# Autodesk Inventor assembly: ModuleBase
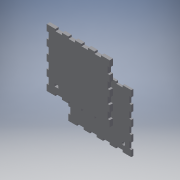
[picture p0: Inventor's stored thumbnail of the model, 180x180]
Saved by Autodesk Inventor 2019.4 (Build 234330000, 330)
## iProperties
Created: 2020-06-30
Part Number: ModuleBase
Document SubType Name: Assembly
Designer: wimva
Author: wimva
## Documents named in this file (4)
- C:\Users\wimva\source\repos\BombSquad\Mechanical\Modules\ModuleBase.iam
- C:\Users\wimva\source\repos\BombSquad\Mechanical\Modules\FrontPlateBase.ipt
- C:\Users\wimva\source\repos\BombSquad\Mechanical\Modules\BackPlateBase.ipt
- C:\Users\wimva\source\repos\BombSquad\Mechanical\Modules\Dimensions.xlsx
## Components (2 placed, 2 different names)
1. FrontPlateBase:1
2. BackPlateBase:1
## Named parameters: RackWidth = 482.6 mm, U = 44.5 mm, ModuleWidth = 96.52 mm, ModuleHeight = 89 mm, ModuleDepth = 50 mm, ModuleCaseThickness = 3 mm, ModuleBottomThickness = 5 mm, ModuleCaseSlotWidth = 10 mm, LaserThickness = 0 mm, ModuleCaseSlotDepth = 3 mm, ModuleConnectorHeight = 6 mm, ModuleConnectorWidth = 6 mm, ModuleConnectorDepth = 4 mm, ModuleConnectorHoleWidth = 6 mm, ModuleConnectorHoleHeight = 4 mm
